# Autodesk Inventor assembly: UpperBody
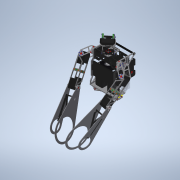
[picture p0: Inventor's stored thumbnail of the model, 180x180]
Saved by Autodesk Inventor 2020.4 (Build 244396000, 396)
## iProperties
Created: 2016-05-03
Part Number: UpperBody
Document SubType Name: Assembly
Designer: hiroaki
Mass: 1684.21 g
Surface Area: 5710.79 cm^2
Volume: 1053.68 cm^3
Density: 1.59841 g/cm^3
Author: hiroaki
## Documents named in this file (9)
- C:\Users\Masato\Documents\Inventor\CIT Brains_Inventor\OpenPlatform_ver3_0 - ve4_1 branch\UpperBody\UpperBody.iam
- C:\Users\Masato\Documents\Inventor\CIT Brains_Inventor\OpenPlatform_ver3_0 - ve4_1 branch\UpperBody\Arm\ForeArm.iam
- C:\Users\Masato\Documents\Inventor\CIT Brains_Inventor\OpenPlatform_ver3_0 - ve4_1 branch\UpperBody\Arm\UpperArm.iam
- C:\Users\Masato\Documents\Inventor\CIT Brains_Inventor\OpenPlatform_ver3_0 - ve4_1 branch\UpperBody\Arm\UpperArm_MIR.iam
- C:\Users\Masato\Documents\Inventor\CIT Brains_Inventor\OpenPlatform_ver3_0 - ve4_1 branch\UpperBody\Head\Head_.iam
- C:\Users\Masato\Documents\Inventor\CIT Brains_Inventor\OpenPlatform_ver3_0 - ve4_1 branch\UpperBody\UpperBody_.iam
- C:\Users\Masato\Documents\Inventor\CIT Brains_Inventor\OpenPlatform_ver3_0 - ve4_1 branch\UpperBody\Cockpit\Cockpit_.iam
- C:\Users\Masato\Documents\Inventor\CIT Brains_Inventor\OpenPlatform_ver3_0 - ve4_1 branch\Ready_Made\Screw\SPNFL-BRN-M3-6.ipt
- C:\Users\Masato\Documents\Inventor\CIT Brains_Inventor\OpenPlatform_ver3_0 - ve4_1 branch\UpperBody\Arm\Shoulder_.iam
## Components (11 placed, 8 different names)
1. ForeArm:1 [sub-assembly] — 挿入:102, 角度:32
2. UpperArm_MIR:1 [sub-assembly] — 挿入:98, 角度:26, 挿入:113, 角度:35
3. ForeArm:2 [sub-assembly] — 挿入:98, 角度:26
4. UpperArm:1 [sub-assembly] — 挿入:102, 角度:32, 挿入:111, 角度:34
5. Head_:1 [sub-assembly] — 挿入:106
6. UpperBody_:1 [sub-assembly] — 挿入:106, フラッシュ:1, フラッシュ:2, フラッシュ:3, 挿入:107, 角度:28, 挿入:108, 挿入:109, 挿入:110, 挿入:112, 角度:36
7. Cockpit_:1 [sub-assembly] — 挿入:107, 角度:28
8. SPNFL-BRN-M3-6:1 — 挿入:108
9. SPNFL-BRN-M3-6:2 — 挿入:109
10. Shoulder_:1 [sub-assembly] — 挿入:110, 挿入:111, 角度:33, 角度:34, 角度:36
11. Shoulder_:2 [sub-assembly] — 挿入:112, 挿入:113, 角度:33, 角度:35
## Relationships (20: Insert 10, Angle 7, Flush 3)
- 挿入:98 [Insert]: UpperArm_MIR:1 ↔ ForeArm:2
- 挿入:102 [Insert]: ForeArm:1 ↔ UpperArm:1
- 角度:26 [Angle] (0 deg): UpperArm_MIR:1 ↔ ForeArm:2
- 挿入:106 [Insert]: Head_:1 ↔ UpperBody_:1
- フラッシュ:1 [Flush]: UpperBody_:1
- フラッシュ:2 [Flush]: UpperBody_:1
- フラッシュ:3 [Flush]: UpperBody_:1
- 挿入:107 [Insert] (0.25 mm): UpperBody_:1 ↔ Cockpit_:1
- 角度:28 [Angle] (0 deg): UpperBody_:1 ↔ Cockpit_:1
- 挿入:108 [Insert]: UpperBody_:1 ↔ SPNFL-BRN-M3-6:1
- 挿入:109 [Insert]: UpperBody_:1 ↔ SPNFL-BRN-M3-6:2
- 角度:32 [Angle] (0 deg): ForeArm:1 ↔ UpperArm:1
- 挿入:110 [Insert]: UpperBody_:1 ↔ Shoulder_:1
- 挿入:111 [Insert]: UpperArm:1 ↔ Shoulder_:1
- 挿入:112 [Insert]: UpperBody_:1 ↔ Shoulder_:2
- 挿入:113 [Insert]: UpperArm_MIR:1 ↔ Shoulder_:2
- 角度:33 [Angle] (0 deg): Shoulder_:1 ↔ Shoulder_:2
- 角度:34 [Angle] (-10 deg): UpperArm:1 ↔ Shoulder_:1
- 角度:35 [Angle] (-10 deg): UpperArm_MIR:1 ↔ Shoulder_:2
- 角度:36 [Angle] (-38.8515 deg): UpperBody_:1 ↔ Shoulder_:1
